# Autodesk Inventor assembly: silnik
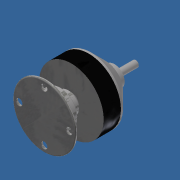
[picture p0: Inventor's stored thumbnail of the model, 180x180]
Saved by Autodesk Inventor 2014 SP1 (Build 180222100, 222)
## iProperties
Created: 2014-09-01
Part Number: silnik
Document SubType Name: Assembly
Designer: Marcin
Author: Marcin
## Documents named in this file (3)
- C:\Users\Marcin\SkyDrive\Dokumenty\Quadrocopter\LabVIEW 3D Model\Silnik\silnik.iam
- C:\Users\Marcin\SkyDrive\Dokumenty\Quadrocopter\LabVIEW 3D Model\Silnik\Podstawa.ipt
- C:\Users\Marcin\SkyDrive\Dokumenty\Quadrocopter\LabVIEW 3D Model\Silnik\Wirnik.ipt
## Components (2 placed, 2 different names)
1. Podstawa:1 — Zestawiający:1, Równoległy:1, Równoległy:2, Równoległy:3
2. Wirnik:1 — Zestawiający:1, Równoległy:1, Równoległy:2
## Relationships (4: Flush 3, Mate 1)
- Zestawiający:1 [Mate]: Podstawa:1 ↔ Wirnik:1
- Równoległy:1 [Flush]: Podstawa:1 ↔ Wirnik:1
- Równoległy:2 [Flush]: Podstawa:1 ↔ Wirnik:1
- Równoległy:3 [Flush]: Podstawa:1
